# Autodesk Inventor assembly: WG18TightBend13mm
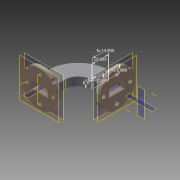
[picture p0: Inventor's stored thumbnail of the model, 180x180]
Saved by Autodesk Inventor 2015 (Build 190159000, 159)
## iProperties
Created: 2014-05-19
Part Number: WG18TightBend13mm
Document SubType Name: Assembly
Designer: jad211
Author: jad211
## Documents named in this file (3)
- C:\CADFiles\EDM Machine\EDM New Pumping Region\WG18TightBend13mm.iam
- C:\CADFiles\EDM Machine\EDM New Pumping Region\WG18FLANGECutDown.ipt
- C:\CADFiles\EDM Machine\EDM New Pumping Region\curved waveguide.ipt
## Components (3 placed, 2 different names)
1. WG18FLANGECutDown:1 — Flush:1, Mate:3, Mate:4, Mate:15, Mate:16, Flush:4
2. WG18FLANGECutDown:2 — Flush:2, Mate:1, Mate:2, Mate:11, Mate:12, Flush:3, Flush:6, Mate:22
3. curved waveguide:1 — Flush:6, Mate:21, Mate:22
## Relationships (29: Mate 22, Flush 6, Angle 1)
- Flush:1: WG18FLANGECutDown:1
- Flush:2: WG18FLANGECutDown:2
- Mate:1: WG18FLANGECutDown:2
- Mate:2: WG18FLANGECutDown:2
- Mate:3: WG18FLANGECutDown:1
- Mate:4: WG18FLANGECutDown:1
- Mate:5
- Mate:6
- Mate:7
- Mate:8
- Mate:9
- Mate:10
- Angle:1 (90 deg)
- Mate:11: WG18FLANGECutDown:2
- Mate:12: WG18FLANGECutDown:2
- Mate:13
- Mate:14
- Mate:15: WG18FLANGECutDown:1
- Mate:16: WG18FLANGECutDown:1
- Mate:17
- Mate:18
- Flush:3: WG18FLANGECutDown:2
- Flush:4: WG18FLANGECutDown:1
- Flush:5 (37 mm)
- Mate:19 (-37 mm)
- Mate:20
- Flush:6: WG18FLANGECutDown:2 ↔ curved waveguide:1
- Mate:21: curved waveguide:1
- Mate:22: WG18FLANGECutDown:2 ↔ curved waveguide:1
